# Autodesk Inventor assembly: Zoetrope
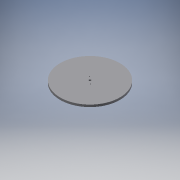
[picture p0: Inventor's stored thumbnail of the model, 180x180]
Saved by Autodesk Inventor 2016 (Build 200138000, 138)
## iProperties
Created: 2019-01-16
Part Number: Zoetrope
Document SubType Name: Assembly
Designer: student
Author: student
## Documents named in this file (4)
- C:\Users\student.MVTHS-ENG-S12\Documents\Nathan_Sneaky_Folder\Zoetrope.iam
- C:\Users\student.MVTHS-ENG-S12\Documents\Nathan_Sneaky_Folder\Zoetrope_Motor_Connector v3.ipt
- C:\Users\student.MVTHS-ENG-S12\Documents\Nathan_Sneaky_Folder\Zoetrope_Motor.ipt
- C:\Users\student.MVTHS-ENG-S12\Documents\Nathan_Sneaky_Folder\Zoetrope_Board.ipt
## Components (3 placed, 3 different names)
1. Zoetrope_Motor_Connector v3:1 — Mate:1, Mate:2, Mate:3, Mate:4, Mate:5
2. Zoetrope_Motor:1 — Mate:1, Mate:2, Mate:3
3. Zoetrope_Board:1 — Mate:4, Mate:5
## Relationships (5: Mate 5)
- Mate:1: Zoetrope_Motor_Connector v3:1 ↔ Zoetrope_Motor:1
- Mate:2: Zoetrope_Motor_Connector v3:1 ↔ Zoetrope_Motor:1
- Mate:3: Zoetrope_Motor_Connector v3:1 ↔ Zoetrope_Motor:1
- Mate:4: Zoetrope_Motor_Connector v3:1 ↔ Zoetrope_Board:1
- Mate:5: Zoetrope_Motor_Connector v3:1 ↔ Zoetrope_Board:1
